# Autodesk Inventor assembly: Ebox_assy
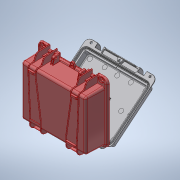
[picture p0: Inventor's stored thumbnail of the model, 180x180]
Saved by Autodesk Inventor 2021 (Build 250183000, 183)
## iProperties
Created: 2021-02-08
Part Number: Ebox_assy
Document SubType Name: Assembly
Designer: Jorian Brusind
Author: Jorian Brusind
## Documents named in this file (5)
- C:\Users\Jorian Brusind\Documents\GitHub\PersonalProjects\HyperRail\Inventor Files\Ebox_assy.iam
- C:\Users\Jorian Brusind\Documents\GitHub\PersonalProjects\HyperRail\Inventor Files\se300-t-b.iam
- C:\Users\Jorian Brusind\Documents\GitHub\PersonalProjects\Inventor Projects\S-201-24.ipt
- C:\Users\Jorian Brusind\Documents\GitHub\PersonalProjects\Inventor Projects\Useful models\Raspberry Pi 3.iam
- C:\Users\Jorian Brusind\Documents\GitHub\PersonalProjects\HyperRail\PCB Files\ESP32 GRBL Controller\ExportSTEP\Main.iam
## Components (4 placed, 4 different names)
1. se300-t-b:1 [sub-assembly] — Mate:9, Mate:10, Mate:11, Mate:21
2. S-201-24:1 — Mate:9, Mate:10, Mate:11, Mate:18, Mate:20, Flush:4, Flush:5, Flush:6
3. Raspberry Pi 3:1 [sub-assembly] — Mate:18, Flush:5, Flush:6
4. Main:1 [sub-assembly] — Mate:20, Mate:21, Flush:4
## Relationships (9: Mate 6, Flush 3)
- Mate:9 (5 mm): se300-t-b:1 ↔ S-201-24:1
- Mate:10: se300-t-b:1 ↔ S-201-24:1
- Mate:11 (5 mm): se300-t-b:1 ↔ S-201-24:1
- Mate:18 (5 mm): S-201-24:1 ↔ Raspberry Pi 3:1
- Mate:20: S-201-24:1 ↔ Main:1
- Mate:21 (30 mm): se300-t-b:1 ↔ Main:1
- Flush:4 (30 mm): S-201-24:1 ↔ Main:1
- Flush:5: S-201-24:1 ↔ Raspberry Pi 3:1
- Flush:6: S-201-24:1 ↔ Raspberry Pi 3:1
